# Autodesk Inventor assembly: Assembly1
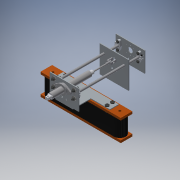
[picture p0: Inventor's stored thumbnail of the model, 180x180]
Saved by Autodesk Inventor 2019 (Build 230136000, 136)
## iProperties
Created: 2021-10-31
Part Number: Assembly1
Document SubType Name: Assembly
Designer: Mohamed Teleb
Author: Mohamed Teleb
## iProperties of the stored document Connector.ipt
Created: 2021-10-31
Part Number: Connector
Material: Generic
Document SubType Name: Modeling
Designer: Mohamed Teleb
Mass: 2.21562 g
Surface Area: 23.0354 cm^2
Volume: 2.21562 cm^3
Density: 1 g/cm^3
Appearance: Default
Author: Mohamed Teleb
## iProperties of the stored document ISO 8738 - 8(2).ipt
Created: 2021-02-02
Part Number: ISO 8738 - 8(2)
Material: Steel
Document SubType Name: Modeling
Designer: Mohamed Teleb
Mass: 1.98525 g
Surface Area: 3.97411 cm^2
Volume: 0.252898 cm^3
Density: 7.85 g/cm^3
Appearance: Default
Author: Mohamed Teleb
## iProperties of the stored document SideToConveyer.ipt
Created: 2021-10-21
Part Number: SideToConveyer
Material: Generic
Document SubType Name: Modeling
Designer: Mohamed Teleb
Mass: 54.5034 g
Surface Area: 351.126 cm^2
Volume: 54.5034 cm^3
Density: 1 g/cm^3
Appearance: Default
Author: Mohamed Teleb
## iProperties of the stored document Pneumatic Cylinder dia 20 L 208 mm.ipt.ipt
Created: 2021-10-31
Part Number: Pneumatic Cylinder dia 20 L 208 mm.ipt
Material: Generic
Document SubType Name: Modeling
Designer: Mohamed Teleb
Mass: 82.4608 g
Surface Area: 181.086 cm^2
Volume: 82.4608 cm^3
Density: 1 g/cm^3
Appearance: Default
Author: Mohamed Teleb
Revision Number: ANY
## iProperties of the stored document ISO 4033 - M6 - ISO.ipt
Created: 2021-02-02
Part Number: ISO 4033 - M6 - ISO
Material: Steel
Document SubType Name: Modeling
Designer: Mohamed Teleb
Mass: 2.90464 g
Surface Area: 3.88882 cm^2
Volume: 0.370018 cm^3
Density: 7.85 g/cm^3
Appearance: Default
Author: Mohamed Teleb
## iProperties of the stored document ISO 14583 - M8x25-4.8.ipt
Created: 2021-02-02
Part Number: ISO 14583 - M8x25-4.8
Material: Steel
Document SubType Name: Modeling
Designer: Mohamed Teleb
Mass: 16.8089 g
Surface Area: 12.8139 cm^2
Volume: 2.14126 cm^3
Density: 7.85 g/cm^3
Appearance: Default
Author: Mohamed Teleb
## iProperties of the stored document PneumaticHolder.ipt
Created: 2021-10-21
Part Number: PneumaticHolder
Material: Generic
Document SubType Name: Modeling
Designer: Mohamed Teleb
Mass: 51.7067 g
Surface Area: 327.844 cm^2
Volume: 51.7067 cm^3
Density: 1 g/cm^3
Appearance: Default
Author: Mohamed Teleb
## iProperties of the stored document GuideRod.ipt
Created: 2021-10-21
Part Number: GuideRod
Material: Generic
Document SubType Name: Modeling
Designer: Mohamed Teleb
Mass: 23.5619 g
Surface Area: 95.8186 cm^2
Volume: 23.5619 cm^3
Density: 1 g/cm^3
Appearance: Default
Author: Mohamed Teleb
## iProperties of the stored document ISO 7045 - M6 x 25_ - 4.8 - H - ISO.ipt
Created: 2021-02-02
Part Number: ISO 7045 - M6 x 25_ - 4.8 - H - ISO
Material: Steel
Document SubType Name: Modeling
Designer: Mohamed Teleb
Mass: 8.35408 g
Surface Area: 8.39982 cm^2
Volume: 1.06421 cm^3
Density: 7.85 g/cm^3
Appearance: Default
Author: Mohamed Teleb
## iProperties of the stored document ISO 7093 A - ST 6 - 140 HV.ipt
Created: 2021-02-02
Part Number: ISO 7093 A - ST 6 - 140 HV
Material: Stainless Steel
Document SubType Name: Modeling
Designer: Mohamed Teleb
Mass: 2.84543 g
Surface Area: 5.67246 cm^2
Volume: 0.355679 cm^3
Density: 8 g/cm^3
Appearance: Default
Author: Mohamed Teleb
## iProperties of the stored document ISO 7092 - ST 6 - 140 HV.ipt
Created: 2021-02-02
Part Number: ISO 7092 - ST 6 - 140 HV
Material: Stainless Steel
Document SubType Name: Modeling
Designer: Mohamed Teleb
Mass: 0.80465 g
Surface Area: 2.13188 cm^2
Volume: 0.100581 cm^3
Density: 8 g/cm^3
Appearance: Default
Author: Mohamed Teleb
## iProperties of the stored document Part1.ipt
Created: 2021-10-21
Part Number: Part1
Material: Generic
Document SubType Name: Modeling
Designer: Mohamed Teleb
Mass: 183.619 g
Surface Area: 465.973 cm^2
Volume: 183.619 cm^3
Density: 1 g/cm^3
Appearance: Default
Author: Mohamed Teleb
## iProperties of the stored document PistonRod.ipt
Created: 2021-10-30
Part Number: PistonRod
Material: Generic
Document SubType Name: Modeling
Designer: Mohamed Teleb
Mass: 3.42918 g
Surface Area: 25.7418 cm^2
Volume: 3.42918 cm^3
Density: 1 g/cm^3
Appearance: Default
Author: Mohamed Teleb
Revision Number: ANY
## iProperties of the stored document BaseForMatlab.iam
Created: 2021-10-31
Part Number: BaseForMatlab
Document SubType Name: Assembly
Designer: Mohamed Teleb
Sending System: Autodesk Inventor 2022
Preprocessor: ST-DEVELOPER v18.1
Title: E:\DesignOfMechatronics1\IndustrialLine\Assembly Module\DOM1STEP\MatlabFiles\BaseForMatlab.stp
Author: Mohamed Teleb
## iProperties of the stored document SHF10.ipt
Created: 2016-08-02
Part Number: SHF10
Material: Generic
Document SubType Name: Modeling
Designer: Mohamed Teleb
Mass: 5.41262 g
Surface Area: 35.7898 cm^2
Volume: 5.41262 cm^3
Density: 1 g/cm^3
Appearance: Default
Author: Mohamed Teleb
## iProperties of the stored document PneumaticHolder.ipt
Created: 2021-10-31
Part Number: PneumaticHolder
Material: Generic
Document SubType Name: Modeling
Designer: Mohamed Teleb
Mass: 13.6143 g
Surface Area: 55.597 cm^2
Volume: 13.6143 cm^3
Density: 1 g/cm^3
Appearance: Default
Author: Mohamed Teleb
## iProperties of the stored document ISO 4034 - M8 - ISO.ipt
Created: 2021-02-02
Part Number: ISO 4034 - M8 - ISO
Material: Steel
Document SubType Name: Modeling
Designer: Mohamed Teleb
Mass: 6.64798 g
Surface Area: 6.8876 cm^2
Volume: 0.846876 cm^3
Density: 7.85 g/cm^3
Appearance: Default
Author: Mohamed Teleb
## iProperties of the stored document Part7.ipt
Created: 2021-10-18
Part Number: Part7
Material: Generic
Document SubType Name: Modeling
Designer: Mohamed Teleb
Mass: 57.2522 g
Surface Area: 1160.31 cm^2
Volume: 57.2522 cm^3
Density: 1 g/cm^3
Appearance: Default
Author: Mohamed Teleb
## iProperties of the stored document StepperHolder.ipt
Created: 2021-10-21
Part Number: StepperHolder
Material: Generic
Document SubType Name: Modeling
Designer: Mohamed Teleb
Mass: 36.9151 g
Surface Area: 243.152 cm^2
Volume: 36.9151 cm^3
Density: 1 g/cm^3
Appearance: Default
Author: Mohamed Teleb
## iProperties of the stored document PneumaticCylinder.iam
Created: 2021-10-31
Part Number: PneumaticCylinder
Document SubType Name: Assembly
Designer: Mohamed Teleb
Sending System: Autodesk Inventor 2022
Preprocessor: ST-DEVELOPER v18.1
Title: E:\DesignOfMechatronics1\IndustrialLine\Assembly Module\DOM1STEP\MatlabFiles\PneumaticCylinder.stp
Author: Mohamed Teleb
## iProperties of the stored document UpperStepperHolder.ipt
Created: 2021-10-21
Part Number: UpperStepperHolder
Material: Generic
Document SubType Name: Modeling
Designer: Mohamed Teleb
Mass: 37.0292 g
Surface Area: 243.838 cm^2
Volume: 37.0292 cm^3
Density: 1 g/cm^3
Appearance: Default
Author: Mohamed Teleb
## Documents named in this file (25)
- **E:\DesignOfMechatronics1\IndustrialLine\Assembly Module\DOM1STEP\MatlabFiles\Assembly1.iam*LocalDocs*xFed3ngmzKf0veqo31etzn5xiEa*Connector.ipt
- **E:\DesignOfMechatronics1\IndustrialLine\Assembly Module\DOM1STEP\MatlabFiles\Assembly1.iam*LocalDocs*xB4ykm2rzWjjaug43Hbdpuq2iZe*ISO 8738 - 8(2).ipt
- **E:\DesignOfMechatronics1\IndustrialLine\Assembly Module\DOM1STEP\MatlabFiles\Assembly1.iam*LocalDocs*x2lqvtbvrX53huuse2gunfyzxXh*SideToConveyer.ipt
- **E:\DesignOfMechatronics1\IndustrialLine\Assembly Module\DOM1STEP\MatlabFiles\Assembly1.iam*LocalDocs*x04vqjdw23tneu3gy41ny1nfo2h*Pneumatic Cylinder dia 20 L 208 mm.ipt.ipt
- **E:\DesignOfMechatronics1\IndustrialLine\Assembly Module\DOM1STEP\MatlabFiles\Assembly1.iam*LocalDocs*xAjldyax5ZspxubobLd1vghiaDh*ISO 4033 - M6 - ISO.ipt
- **E:\DesignOfMechatronics1\IndustrialLine\Assembly Module\DOM1STEP\MatlabFiles\Assembly1.iam*LocalDocs*xE1dwgdv2P0vzutwg2te4u11yEe*ISO 14583 - M8x25-4.8.ipt
- **E:\DesignOfMechatronics1\IndustrialLine\Assembly Module\DOM1STEP\MatlabFiles\Assembly1.iam*LocalDocs*xDnza0q5aCaqqubsmLv0bw4xdNg*PneumaticHolder.ipt
- **E:\DesignOfMechatronics1\IndustrialLine\Assembly Module\DOM1STEP\MatlabFiles\Assembly1.iam*LocalDocs*xEjkofyejQpvuuhw0Ze2ox1sm1e*GuideRod.ipt
- **E:\DesignOfMechatronics1\IndustrialLine\Assembly Module\DOM1STEP\MatlabFiles\Assembly1.iam*LocalDocs*xKtaiszha1ya1ei0qCyz0ozehSh*ISO 7045 - M6 x 25_ - 4.8 - H - ISO.ipt
- **E:\DesignOfMechatronics1\IndustrialLine\Assembly Module\DOM1STEP\MatlabFiles\Assembly1.iam*LocalDocs*xGtnz0xj4Jlteua0k1zgoxgt1Cc*ISO 7093 A - ST 6 - 140 HV.ipt
- **E:\DesignOfMechatronics1\IndustrialLine\Assembly Module\DOM1STEP\MatlabFiles\Assembly1.iam*LocalDocs*xGm0jpcmbLrw4erkyBkg0v3j1Cf*ISO 7092 - ST 6 - 140 HV.ipt
- **E:\DesignOfMechatronics1\IndustrialLine\Assembly Module\DOM1STEP\MatlabFiles\Assembly1.iam*LocalDocs*xKiwoaylpTr03eqk1OyfxvqraYb*Part1.ipt
- **E:\DesignOfMechatronics1\IndustrialLine\Assembly Module\DOM1STEP\MatlabFiles\Assembly1.iam*LocalDocs*xQxqzg3ioAnfferopNuygnlfcMf*PistonRod.ipt
- **E:\DesignOfMechatronics1\IndustrialLine\Assembly Module\DOM1STEP\MatlabFiles\Assembly1.iam*LocalDocs*xQ0lx2fitAzbzut4pGnzw55dkBh*BaseForMatlab.iam
- **E:\DesignOfMechatronics1\IndustrialLine\Assembly Module\DOM1STEP\MatlabFiles\Assembly1.iam*LocalDocs*xSm0ardgoHzwsel0oBft0xh5m5e*Part7.ipt
- **E:\DesignOfMechatronics1\IndustrialLine\Assembly Module\DOM1STEP\MatlabFiles\Assembly1.iam*LocalDocs*xU10uzzid3rgkeigzQq22nsjxZc*ISO 4034 - M8 - ISO.ipt
- **E:\DesignOfMechatronics1\IndustrialLine\Assembly Module\DOM1STEP\MatlabFiles\Assembly1.iam*LocalDocs*xWtgdlekfIsjfud0wXvmkfeew1b*StepperHolder.ipt
- **E:\DesignOfMechatronics1\IndustrialLine\Assembly Module\DOM1STEP\MatlabFiles\Assembly1.iam*LocalDocs*xNs2h3cqp1mhwegwqVcsj5qjdPf*SHF10.ipt
- **E:\DesignOfMechatronics1\IndustrialLine\Assembly Module\DOM1STEP\MatlabFiles\Assembly1.iam*LocalDocs*xXrysqutqG5dxuncuIedw0r1hXd*UpperStepperHolder.ipt
- **E:\DesignOfMechatronics1\IndustrialLine\Assembly Module\DOM1STEP\MatlabFiles\Assembly1.iam*LocalDocs*xQc2v52hvAsj2ehs2Wodd11keOh*PneumaticHolder.ipt
- Pneumatic Cylinder dia 20 L 208 mm.ipt
- **E:\DesignOfMechatronics1\IndustrialLine\Assembly Module\DOM1STEP\MatlabFiles\Assembly1.iam*LocalDocs*xUnb4esw45v4ouzciVqmxiw0i3e*PneumaticCylinder.iam
- E:\DesignOfMechatronics1\IndustrialLine\Assembly Module\DOM1STEP\MatlabFiles\Assembly1.iam
- E:\DesignOfMechatronics1\IndustrialLine\Assembly Module\DOM1STEP\MatlabFiles\BaseForMatlab.stp
- E:\DesignOfMechatronics1\IndustrialLine\Assembly Module\DOM1STEP\MatlabFiles\PneumaticCylinder.stp
## Components (2 placed, 2 different names)
1. BaseForMatlab:1 [sub-assembly] — Mate:1, Mate:2
2. PneumaticCylinder:1 [sub-assembly] — Mate:1, Mate:2
## Relationships (2: Mate 2)
- Mate:1: BaseForMatlab:1 ↔ PneumaticCylinder:1
- Mate:2: BaseForMatlab:1 ↔ PneumaticCylinder:1
